# Autodesk Inventor assembly: Finger Assembly Right
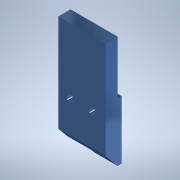
[picture p0: Inventor's stored thumbnail of the model, 180x180]
Saved by Autodesk Inventor 2022 (Build 260153000, 153)
## iProperties
Created: 2021-09-24
Part Number: Finger Assembly Right
Document SubType Name: Assembly
Designer: kylem
Author: kylem
## Documents named in this file (3)
- C:\Users\kylem\OneDrive\Documents\GitHub\IMML_Contactile_Gripper_Hardware\Finger Assembly Right.iam
- C:\Users\kylem\OneDrive\Documents\GitHub\IMML_Contactile_Gripper_Hardware\Contactile Sensor.ipt
- C:\Users\kylem\OneDrive\Documents\GitHub\IMML_Contactile_Gripper_Hardware\Finger_right.ipt
## Components (2 placed, 2 different names)
1. Contactile Sensor:1 — Mate:1, Flush:1, Mate:2
2. Finger_right:1 — Mate:1, Flush:1, Mate:2
## Relationships (3: Mate 2, Flush 1)
- Mate:1: Contactile Sensor:1 ↔ Finger_right:1
- Flush:1: Contactile Sensor:1 ↔ Finger_right:1
- Mate:2: Contactile Sensor:1 ↔ Finger_right:1
